# Autodesk Inventor assembly: ASY MSC 300.2 LEFT BOARD
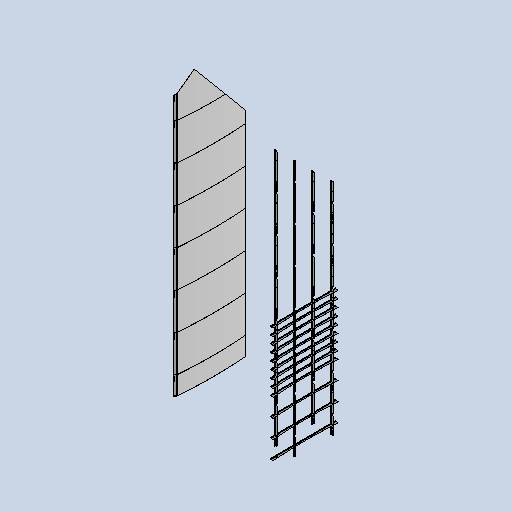
[picture p0: Inventor's stored thumbnail of the model, 512x512]
Saved by Autodesk Inventor 2025 (Build 290162010, 162A)
## iProperties
Created: 2024-07-21
Part Number: ASY MSC 300.2 LEFT BOARD
Document SubType Name: Assembly
Designer: pokla
Stock Number: ASY МОО 300.2 левый борт
Author: pokla
## Documents named in this file (10)
- C:\Users\pokla\Documents\Inventor\Отстойник осветлитель\Manturovo_Se-clar-Gleb\ASY MSC 202 LEFT BOARD.iam
- C:\Users\pokla\Documents\Inventor\Отстойник осветлитель\Manturovo_Se-clar-Gleb\MSC 305 RIB BOARD.ipt
- C:\Users\pokla\Documents\Inventor\Отстойник осветлитель\Manturovo_Se-clar-Gleb\MSC 024 sheet board main.ipt
- C:\Users\pokla\Documents\Inventor\Отстойник осветлитель\Manturovo_Se-clar-Gleb\MSC 023 sheet board.ipt
- C:\Users\pokla\Documents\Inventor\Отстойник осветлитель\Manturovo_Se-clar-Gleb\MSC 025 sheet board withers 1.ipt
- C:\Users\pokla\Documents\Inventor\Отстойник осветлитель\Manturovo_Se-clar-Gleb\MSC 027 sheet board face 1.ipt
- C:\Users\pokla\Documents\Inventor\Отстойник осветлитель\Manturovo_Se-clar-Gleb\MSC 306 stringer BOARD  #.ipt
- C:\Users\pokla\Documents\Inventor\Отстойник осветлитель\Manturovo_Se-clar-Gleb\MSC 307 stringer BOARD  ##.ipt
- C:\Users\pokla\Documents\Inventor\Отстойник осветлитель\Manturovo_Se-clar-Gleb\MSC 308 stringer BOARD  ###.ipt
- C:\Users\pokla\Documents\Inventor\Отстойник осветлитель\Manturovo_Se-clar-Gleb\MSC 309 stringer BOARD  ####.ipt
## Components (46 placed, 9 different names)
1. MSC 023 sheet board.ipt:1 — Mate:2, Rigid:20, Flush:5, Flush:6, Flush:7
2. MSC 024 sheet board main.ipt:1 — Rigid:20, Rigid:21
3. MSC 024 sheet board main.ipt:2 — Rigid:21, Rigid:22
4. MSC 024 sheet board main.ipt:3 — Rigid:22, Rigid:23
5. MSC 024 sheet board main.ipt:4 — Rigid:23, Rigid:24
6. MSC 024 sheet board main.ipt:5 — Rigid:24, Rigid:25
7. MSC 025 sheet board withers 1.ipt:1 — Rigid:25, Rigid:26
8. MSC 027 sheet board face 1.ipt:1 — Rigid:26
9. MSC 052 rib board.ipt:1
10. MSC 052 rib board.ipt:2
11. MSC 306 stringer BOARD  #.ipt:1
12. MSC 307 stringer BOARD  ##.ipt:1
13. MSC 052 rib board.ipt:3
14. MSC 308 stringer BOARD  ###.ipt:1
15. MSC 309 stringer BOARD  ####.ipt:1
16. MSC 309 stringer BOARD  ####.ipt:2
17. MSC 308 stringer BOARD  ###.ipt:2
18. MSC 052 rib board.ipt:4
19. MSC 052 rib board.ipt:5
20. MSC 052 rib board.ipt:6
21. MSC 052 rib board.ipt:7
22. MSC 052 rib board.ipt:8
23. MSC 052 rib board.ipt:9
24. MSC 052 rib board.ipt:10
25. MSC 052 rib board.ipt:11
26. MSC 052 rib board.ipt:12
27. MSC 308 stringer BOARD  ###.ipt:3
28. MSC 309 stringer BOARD  ####.ipt:3
29. MSC 307 stringer BOARD  ##.ipt:2
30. MSC 306 stringer BOARD  #.ipt:2
31. MSC 308 stringer BOARD  ###.ipt:4
32. MSC 309 stringer BOARD  ####.ipt:4
33. MSC 307 stringer BOARD  ##.ipt:3
34. MSC 306 stringer BOARD  #.ipt:3
35. MSC 308 stringer BOARD  ###.ipt:5
36. MSC 309 stringer BOARD  ####.ipt:5
37. MSC 307 stringer BOARD  ##.ipt:4
38. MSC 306 stringer BOARD  #.ipt:4
39. MSC 308 stringer BOARD  ###.ipt:6
40. MSC 309 stringer BOARD  ####.ipt:6
41. MSC 307 stringer BOARD  ##.ipt:5
42. MSC 306 stringer BOARD  #.ipt:5
43. MSC 308 stringer BOARD  ###.ipt:7
44. MSC 309 stringer BOARD  ####.ipt:7
45. MSC 307 stringer BOARD  ##.ipt:6
46. MSC 306 stringer BOARD  #.ipt:6
## Component patterns: (9 elements, first: MSC 052 rib board.ipt:4), (5 elements, first: MSC 308 stringer BOARD  ###.ipt:3 + MSC 309 stringer BOARD  ####.ipt:3 + MSC 307 stringer BOARD  ##.ipt:2 + MSC 306 stringer BOARD  #.ipt:2)
## Relationships (24: WeldJoint 20, Flush 3, Mate 1)
- Mate:2: MSC 023 sheet board.ipt:1
- Rigid:20 [WeldJoint]: MSC 023 sheet board.ipt:1 ↔ MSC 024 sheet board main.ipt:1
- Rigid:21 [WeldJoint]: MSC 024 sheet board main.ipt:1 ↔ MSC 024 sheet board main.ipt:2
- Rigid:22 [WeldJoint]: MSC 024 sheet board main.ipt:2 ↔ MSC 024 sheet board main.ipt:3
- Rigid:23 [WeldJoint]: MSC 024 sheet board main.ipt:3 ↔ MSC 024 sheet board main.ipt:4
- Rigid:24 [WeldJoint]: MSC 024 sheet board main.ipt:4 ↔ MSC 024 sheet board main.ipt:5
- Rigid:25 [WeldJoint]: MSC 024 sheet board main.ipt:5 ↔ MSC 025 sheet board withers 1.ipt:1
- Flush:5: MSC 023 sheet board.ipt:1
- Flush:6: MSC 023 sheet board.ipt:1
- Flush:7: MSC 023 sheet board.ipt:1
- Rigid:26 [WeldJoint]: MSC 025 sheet board withers 1.ipt:1 ↔ MSC 027 sheet board face 1.ipt:1
- [WeldJoint]: MSC 306 stringer BOARD  #.ipt:1 ↔ MSC 306 stringer BOARD  #.ipt:2
- [WeldJoint]: MSC 307 stringer BOARD  ##.ipt:1 ↔ MSC 307 stringer BOARD  ##.ipt:2
- [WeldJoint]: MSC 308 stringer BOARD  ###.ipt:1 ↔ MSC 308 stringer BOARD  ###.ipt:2
- [WeldJoint]: MSC 308 stringer BOARD  ###.ipt:1 ↔ MSC 308 stringer BOARD  ###.ipt:3
- [WeldJoint]: MSC 309 stringer BOARD  ####.ipt:1 ↔ MSC 309 stringer BOARD  ####.ipt:2
- [WeldJoint]: MSC 309 stringer BOARD  ####.ipt:1 ↔ MSC 309 stringer BOARD  ####.ipt:3
- [WeldJoint] (2 mm): MSC 052 rib board.ipt:2 ↔ MSC 306 stringer BOARD  #.ipt:1
- [WeldJoint] (2 mm): MSC 052 rib board.ipt:3 ↔ MSC 306 stringer BOARD  #.ipt:2
- [WeldJoint] (2 mm): MSC 052 rib board.ipt:4 ↔ MSC 306 stringer BOARD  #.ipt:2
- [WeldJoint] (2 mm): MSC 052 rib board.ipt:2 ↔ MSC 309 stringer BOARD  ####.ipt:2
- [WeldJoint] (2 mm): MSC 052 rib board.ipt:2 ↔ MSC 307 stringer BOARD  ##.ipt:1
- [WeldJoint] (2 mm): MSC 052 rib board.ipt:2 ↔ MSC 308 stringer BOARD  ###.ipt:2
- [WeldJoint] (2 mm): MSC 052 rib board.ipt:1 ↔ MSC 306 stringer BOARD  #.ipt:1
